# Autodesk Inventor assembly: ShoulderLeft
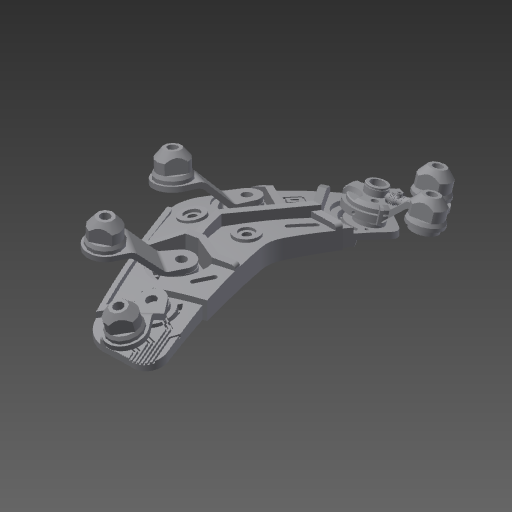
[picture p0: Inventor's stored thumbnail of the model, 512x512]
Saved by Autodesk Inventor 2020 (Build 240168000, 168)
## iProperties
Created: 2016-10-02
Part Number: ShoulderLeft
Document SubType Name: Assembly
Designer: Val
Author: Val
## Documents named in this file (8)
- C:\Users\valer\Desktop\elysium-max-exoskeleton\src\Assemblies\ShoulderRight.iam
- C:\Users\valer\Desktop\elysium-max-exoskeleton\src\ShoulderCogLarge.ipt
- C:\Users\valer\Desktop\elysium-max-exoskeleton\src\ShoulderCogSmall.ipt
- C:\Users\valer\Desktop\elysium-max-exoskeleton\src\BackConnector.ipt
- C:\Users\valer\Desktop\elysium-max-exoskeleton\src\BackSideConnector.ipt
- C:\Users\valer\Desktop\elysium-max-exoskeleton\src\Assemblies\ShoulderConnector.iam
- C:\Users\valer\Desktop\elysium-max-exoskeleton\src\ShoulderRight.ipt
- C:\Users\valer\Desktop\elysium-max-exoskeleton\src\SpacerShort.ipt
## Components (15 placed, 7 different names)
1. ShoulderCogLarge:1 — Mate:19, Mate:20, Mate:22
2. ShoulderCogSmall:1 — Mate:14, Mate:29, Mate:30, Mate:31
3. ShoulderCogSmall:2 — Mate:16, Mate:26, Mate:27
4. ShoulderCogSmall:3 — Mate:18, Mate:23, Mate:24
5. BackConnector:1 — Mate:14, Mate:31, Mate:32, Mate:41, Mate:42
6. BackSideConnector:1 — Mate:11, Mate:12, Mate:33, Mate:34, Mate:36
7. BackConnector:2 — Mate:16, Mate:28, Mate:39, Mate:40
8. BackConnector:3 — Mate:18, Mate:25, Mate:37, Mate:38
9. ShoulderConnectorSplit:1 [sub-assembly] — Mate:11, Mate:12, Mate:21, Mate:22, Mate:35
10. ShoulderRight:1 — Mate:19, Mate:20, Mate:21, Mate:23, Mate:24, Mate:25, Mate:26, Mate:27, Mate:28, Mate:29, Mate:30, Mate:32
11. SpacerShort:1 — Mate:33, Mate:35
12. SpacerShort:2 — Mate:34, Mate:36
13. SpacerShort:3 — Mate:37, Mate:38
14. SpacerShort:4 — Mate:39, Mate:40
15. SpacerShort:5 — Mate:41, Mate:42
## Relationships (29: Mate 29)
- Mate:11: BackSideConnector:1 ↔ ShoulderConnectorSplit:1
- Mate:12: BackSideConnector:1 ↔ ShoulderConnectorSplit:1
- Mate:14: ShoulderCogSmall:1 ↔ BackConnector:1
- Mate:16: ShoulderCogSmall:2 ↔ BackConnector:2
- Mate:18: ShoulderCogSmall:3 ↔ BackConnector:3
- Mate:19: ShoulderCogLarge:1 ↔ ShoulderRight:1
- Mate:20: ShoulderCogLarge:1 ↔ ShoulderRight:1
- Mate:21: ShoulderConnectorSplit:1 ↔ ShoulderRight:1
- Mate:22: ShoulderCogLarge:1 ↔ ShoulderConnectorSplit:1
- Mate:23: ShoulderCogSmall:3 ↔ ShoulderRight:1
- Mate:24: ShoulderCogSmall:3 ↔ ShoulderRight:1
- Mate:25: BackConnector:3 ↔ ShoulderRight:1
- Mate:26: ShoulderCogSmall:2 ↔ ShoulderRight:1
- Mate:27: ShoulderCogSmall:2 ↔ ShoulderRight:1
- Mate:28: BackConnector:2 ↔ ShoulderRight:1
- Mate:29: ShoulderCogSmall:1 ↔ ShoulderRight:1
- Mate:30: ShoulderCogSmall:1 ↔ ShoulderRight:1
- Mate:31: ShoulderCogSmall:1 ↔ BackConnector:1
- Mate:32: BackConnector:1 ↔ ShoulderRight:1
- Mate:33: BackSideConnector:1 ↔ SpacerShort:1
- Mate:34: BackSideConnector:1 ↔ SpacerShort:2
- Mate:35: ShoulderConnectorSplit:1 ↔ SpacerShort:1
- Mate:36: BackSideConnector:1 ↔ SpacerShort:2
- Mate:37: BackConnector:3 ↔ SpacerShort:3
- Mate:38: BackConnector:3 ↔ SpacerShort:3
- Mate:39: BackConnector:2 ↔ SpacerShort:4
- Mate:40: BackConnector:2 ↔ SpacerShort:4
- Mate:41: BackConnector:1 ↔ SpacerShort:5
- Mate:42: BackConnector:1 ↔ SpacerShort:5
